# Autodesk Inventor assembly: 8-inch_Skid
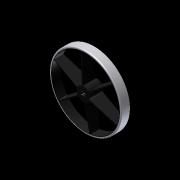
[picture p0: Inventor's stored thumbnail of the model, 180x180]
Saved by Autodesk Inventor 2011 SP1 (Build 150282100, 282)
## iProperties
Created: 2013-01-14
Part Number: 8-inch_Skid
Document SubType Name: Assembly
Designer: 939551
Author: 939551
## Documents named in this file (3)
- \\WW427-DATA1\StuHome\939551\Documents\GitHub\2013CAD\8-inch_Skid.iam
- \\WW427-DATA1\StuHome\939551\Documents\GitHub\2013CAD\Wheel_Rim.ipt
- \\WW427-DATA1\StuHome\939551\Documents\GitHub\2013CAD\Wheel_Spokes.ipt
## Components (2 placed, 2 different names)
1. Wheel_Rim:1 — Insert:1, Rotation:1, Insert:2
2. Wheel_Spokes:1 — Insert:1, Rotation:1, Insert:2
## Relationships (3: Insert 2, RelateRotation 1)
- Insert:1: Wheel_Rim:1 ↔ Wheel_Spokes:1
- Rotation:1 [RelateRotation] (1 ul): Wheel_Rim:1 ↔ Wheel_Spokes:1
- Insert:2: Wheel_Rim:1 ↔ Wheel_Spokes:1
